# Autodesk Inventor assembly: B6201ZZNR
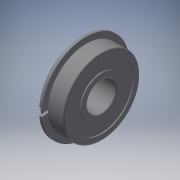
[picture p0: Inventor's stored thumbnail of the model, 180x180]
Saved by Autodesk Inventor 2019 (Build 230136000, 136)
## iProperties
Category: PARTsolutions
Company: MISUMI
Created: 2023-12-27
Part Number: B6201ZZNR
Catalog Web Link: www.cadenas.de
Description: B6_ _ _ZZNR, SB6_ _ _ZZNR-Deep Groove Ball Bearings - Double Shielded with Retaining Ring
Vendor: MISUMI
Document SubType Name: Assembly
Designer: psAdmin
Manufacturer: MISUMI
Mass: 6.86438 g
Surface Area: 38.9985 cm^2
Volume: 6.86438 cm^3
Density: 1 g/cm^3
Title: B6201ZZNR
Author: Cadenas PARTsolutions
Comments: Deep Groove Ball Bearings - Double Shielded with Retaining Ring
PSOL_IDENT_0: {$CADENAS_DATA/23d-libs/misumi/metric/12_bearing_holders/sb6905zznr_asmtab.prj},185 {VTYP=3D},{STYP=
PSOL_IDENT_1: ASSTAB},{NB=B6201ZZNR},{LINA=B6201ZZNR},{NN=B6_ _ _ZZNR, SB6_ _ _ZZNR},{DATE=03.06.2021 05:36:52},{G
PSOL_IDENT_2: EOMDATE=08.09.2011},{VERSION=},{LINEID=100},{WBVAR=TS},{WBNUMERIC=}  {NB=B6201ZZNR},{LINA=B6201ZZNR}
PSOL_IDENT_3: ,{KT=DUMMY},{PN=B6201ZZNR},{TYS=NR},{TS=},{TS1= '', 'Steel', 'S', 'Stainless Steel'},{MAT=52100 Bear
PSOL_IDENT_4: ing Steel},{BN=6201ZZ},{DD=12},{D=32},{B=10},{RR=0.6},{RR1=0.6},{CR=6.80},{COR=3.05},{CRS=6.80},{CRS
PSOL_IDENT_5: S=6.80},{CORS=3.05},{CORSS=3.05},{AA=2.06},{BB=1.35},{D1=36.7},{RR2=0.6},{D2=36.7},{FF=1.12},{DD1=30
PSOL_IDENT_6: .150},{R1=0.400},{R2=0.500},{DSMIN=16.0},{DSMAX=17.0},{DDHH=28.0},{R=0.6},{DX=37.5},{CY=2.9},{CZ=1.2
PSOL_IDENT_7: },{MASS=37},{PPATH=b6700zz_templ.prj}
NB: B6201ZZNR
NN: B6_ _ _ZZNR, SB6_ _ _ZZNR
NT: Deep Groove Ball Bearings - Double Shielded with Retaining Ring
NBSYN: $PN.
LINA: B6201ZZNR
CATALOG: Misumi
PN: B6201ZZNR
TS: Steel
MAT: 52100 Bearing Steel
BN: 6201ZZ
DD: 12
D: 32
B: 10
RR: 0.6
RR1: 0.6
CR: 6.80
COR: 3.05
D1: 36.7
FF: 1.12
DSMIN: 16
DSMAX: 17
DDHH: 28
R: 0.6
DX: 37.5
CY: 2.9
CZ: 1.2
MASS: 37
SUPPLIER: MISUMI
ARTICLENO: B6201ZZNR
BOMINFO: B6201ZZNR
CREATOR: CADENAS GmbH
## Documents named in this file (3)
- e:\temp\worker_COMMON_2\temp\tmp_4420_118_vvR0Z\format_0\B6201ZZNR.iam
- e:\temp\worker_COMMON_2\temp\tmp_4420_118_vvR0Z\format_0\bearingB6201ZZNR.ipt
- e:\temp\worker_COMMON_2\temp\tmp_4420_118_vvR0Z\format_0\RING-6201ZZ.ipt
## Components (2 placed, 2 different names)
1. bearingB6201ZZNR:1 — to_ring_XY@1 <-> ring_to_bearing_XY@2, to_ring_Z@1 <-> ring_to_bearing_Z@2
2. RING-6201ZZ:1 — to_ring_XY@1 <-> ring_to_bearing_XY@2, to_ring_Z@1 <-> ring_to_bearing_Z@2
## Relationships (2: Flush 1, Mate 1)
- to_ring_XY@1 <-> ring_to_bearing_XY@2 [Flush]: bearingB6201ZZNR:1 ↔ RING-6201ZZ:1
- to_ring_Z@1 <-> ring_to_bearing_Z@2 [Mate]: bearingB6201ZZNR:1 ↔ RING-6201ZZ:1
